# Autodesk Inventor assembly: Paper-holder
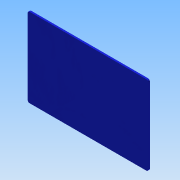
[picture p0: Inventor's stored thumbnail of the model, 180x180]
Saved by Autodesk Inventor 2016 (Build 200138000, 138)
## iProperties
Created: 2015-10-22
Part Number: Paper-holder
Document SubType Name: Assembly
Designer: Openlab
Author: Openlab
## Documents named in this file (4)
- E:\Alex\DI-Lambda\parts\Common\Paper-holder.iam
- E:\Alex\DI-Lambda\parts\Common\Paper-holder-clip.ipt
- E:\Alex\DI-Lambda\parts\Common\Paper-holder.ipt
- E:\Alex\DI-Lambda\parts\Common\A4-paper.ipt
## Components (3 placed, 3 different names)
1. Paper-holder-clip:1 — Mate:2, Flush:3
2. Paper-holder:1 — Mate:2, Mate:3, Flush:1, Flush:2, Flush:3
3. A4-paper:1 — Mate:3, Flush:1, Flush:2
## Relationships (5: Flush 3, Mate 2)
- Mate:2: Paper-holder-clip:1 ↔ Paper-holder:1
- Mate:3: Paper-holder:1 ↔ A4-paper:1
- Flush:1 (10 mm): Paper-holder:1 ↔ A4-paper:1
- Flush:2 (10 mm): Paper-holder:1 ↔ A4-paper:1
- Flush:3 (75 mm): Paper-holder-clip:1 ↔ Paper-holder:1
